# Autodesk Inventor assembly: Cylinder Complete
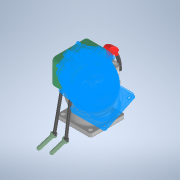
[picture p0: Inventor's stored thumbnail of the model, 180x180]
Saved by Autodesk Inventor 2021 (Build 250183000, 183)
## iProperties
Created: 2022-11-09
Part Number: Cylinder Complete
Document SubType Name: Assembly
Designer: peris
Author: peris
## Documents named in this file (10)
- D:\Inventor\Radial_Engine\Assembly\Cylinder Complete.iam
- D:\Inventor\Radial_Engine\Component 4.ipt
- D:\Inventor\Radial_Engine\Component 39.ipt
- D:\Inventor\Radial_Engine\Component 45.ipt
- D:\Inventor\Radial_Engine\Component 48.ipt
- D:\Inventor\Radial_Engine\Assembly\cylinder sub-assembly.iam
- D:\Inventor\Radial_Engine\Assembly\Rocker Arm subassembly.iam
- D:\Inventor\Radial_Engine\Assembly\valve sub-assembly.iam
- D:\Inventor\Radial_Engine\Component 27.ipt
- D:\Inventor\Radial_Engine\Component 36.ipt
## Components (13 placed, 9 different names)
1. Component 4:1 — Tangent:2
2. Component 39:1 — Tangent:2, Tangent:4
3. Component 4:2 — Tangent:1
4. Component 39:2 — Tangent:1, Tangent:3
5. Component 48:2 — Mate:1, Mate:2
6. cylinder sub-assembly:1 [sub-assembly] — Flush:1, Flush:2, Flush:3, Mate:3, Mate:4, Mate:5, Mate:6, Mate:7, Mate:8, Mate:9, Mate:10, Mate:11, Mate:14, Mate:15, Mate:16, Mate:17, Mate:18
7. Rocker Arm subassembly:1 [sub-assembly] — Mate:8, Mate:10, Tangent:3
8. valve sub-assembly:1 [sub-assembly] — Mate:6, Mate:7
9. Rocker Arm subassembly:2 [sub-assembly] — Mate:9, Mate:11, Tangent:4
10. valve sub-assembly:2 [sub-assembly] — Mate:4, Mate:5
11. Component 45:1 — Mate:1, Mate:2, Mate:3
12. Component 27:1 — Mate:12, Mate:13, Flush:4, Mate:18
13. Component 36:1 — Mate:12, Mate:13, Flush:4, Mate:14, Mate:15, Mate:16, Mate:17
## Relationships (26: Mate 18, Flush 4, Tangent 4)
- Flush:1: cylinder sub-assembly:1
- Flush:2: cylinder sub-assembly:1
- Flush:3: cylinder sub-assembly:1
- Mate:1: Component 48:2 ↔ Component 45:1
- Mate:2: Component 48:2 ↔ Component 45:1
- Mate:3: cylinder sub-assembly:1 ↔ Component 45:1
- Mate:4: cylinder sub-assembly:1 ↔ valve sub-assembly:2
- Mate:5: cylinder sub-assembly:1 ↔ valve sub-assembly:2
- Mate:6: cylinder sub-assembly:1 ↔ valve sub-assembly:1
- Mate:7: cylinder sub-assembly:1 ↔ valve sub-assembly:1
- Mate:8: cylinder sub-assembly:1 ↔ Rocker Arm subassembly:1
- Mate:9: cylinder sub-assembly:1 ↔ Rocker Arm subassembly:2
- Mate:10: cylinder sub-assembly:1 ↔ Rocker Arm subassembly:1
- Mate:11: cylinder sub-assembly:1 ↔ Rocker Arm subassembly:2
- Tangent:1: Component 4:2 ↔ Component 39:2
- Tangent:2: Component 4:1 ↔ Component 39:1
- Tangent:3: Component 39:2 ↔ Rocker Arm subassembly:1
- Tangent:4: Component 39:1 ↔ Rocker Arm subassembly:2
- Mate:12: Component 27:1 ↔ Component 36:1
- Mate:13: Component 27:1 ↔ Component 36:1
- Flush:4: Component 27:1 ↔ Component 36:1
- Mate:14: cylinder sub-assembly:1 ↔ Component 36:1
- Mate:15: cylinder sub-assembly:1 ↔ Component 36:1
- Mate:16: cylinder sub-assembly:1 ↔ Component 36:1
- Mate:17: cylinder sub-assembly:1 ↔ Component 36:1
- Mate:18: cylinder sub-assembly:1 ↔ Component 27:1
